# Autodesk Inventor assembly: Final Mold Assy
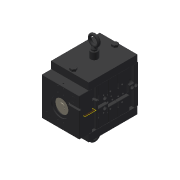
[picture p0: Inventor's stored thumbnail of the model, 180x180]
Saved by Autodesk Inventor 2022 Beta2 (Build 260130000, 130) ContinuousBuild 0
## iProperties
Shininess: 64.0
Length Units: 11269
Angle Units: 11279
Time Units: 11290
Mass Units: 11283
Length Display Precision: 3
Angle Display Precision: 2
Compacted: True
Part Number: Final Mold Assy
Document SubType Name: Assembly
Created: 2003-04-07
Designer: demo
Density: 0.0
Volumn: 0.0
Area: 0.0
PropertySet Name: Model Information
Control State: 0
Master: False
Checked Out: False
Author: demo
## Documents named in this file (9)
- C:\Autodesk Inventor 2021 Intro Practice Files\Mold Assembly\Final Mold Assy.iam
- C:\Autodesk Inventor 2021 Intro Practice Files\Mold Assembly\local.ANSI.62.230.1.ipt
- C:\Autodesk Inventor 2021 Intro Practice Files\Mold Assembly\topplate2 Assy.iam
- C:\Autodesk Inventor 2021 Intro Practice Files\Mold Assembly\Middleplate Assy.iam
- C:\Autodesk Inventor 2021 Intro Practice Files\Mold Assembly\Bottomplate2 assy1.iam
- C:\Autodesk Inventor 2021 Intro Practice Files\Mold Assembly\bottomplate.ipt
- C:\Autodesk Inventor 2021 Intro Practice Files\Mold Assembly\topplate Assy.iam
- C:\Autodesk Inventor 2021 Intro Practice Files\Mold Assembly\Sideplate.ipt
- C:\Autodesk Inventor 2021 Intro Practice Files\Mold Assembly\Grip handle.ipt
## Components (13 placed, 8 different names)
1. topplate2 Assy:1 [sub-assembly] — Mate:1, Flush:1, Mate:2, Flush:5, Flush:6, Mate:6
2. Middleplate Assy:1 [sub-assembly] — Mate:1, Flush:1, Mate:2, Flush:2, Mate:4, Mate:7, Mate:9, Flush:12
3. Bottomplate2 assy1:1 [sub-assembly] — Flush:2, Mate:4, Flush:3, Flush:4, Mate:5, Flush:12
4. topplate Assy:1 [sub-assembly] — Flush:5, Flush:6, Mate:6, Flush:7, Mate:8, Flush:9, Mate:10, Flush:10
5. Sideplate:1 — Mate:7, Flush:7, Flush:8, Mate:8, Mate:11, Insert:1, Insert:3, Insert:4
6. Grip handle:1 — Flush:8, Mate:11, Insert:1, Flush:10
7. Sideplate:2 — Mate:9, Flush:9, Mate:10, Insert:2, Flush:11, Insert:5, Insert:6
8. Grip handle:2 — Insert:2, Flush:11
9. Heavy Hex Bolt - UNC (Regular Thread - Inch) 5/8-11 UNC - 2.5:1 — Insert:3
10. Heavy Hex Bolt - UNC (Regular Thread - Inch) 5/8-11 UNC - 2.5:2 — Insert:4
11. Heavy Hex Bolt - UNC (Regular Thread - Inch) 5/8-11 UNC - 2.5:3 — Insert:5
12. Heavy Hex Bolt - UNC (Regular Thread - Inch) 5/8-11 UNC - 2.5:4 — Insert:6
13. bottomplate:1 — Flush:3, Flush:4, Mate:5
## Relationships (28: Flush 12, Mate 10, Insert 6)
- Mate:1: topplate2 Assy:1 ↔ Middleplate Assy:1
- Flush:1: topplate2 Assy:1 ↔ Middleplate Assy:1
- Mate:2: topplate2 Assy:1 ↔ Middleplate Assy:1
- Flush:2: Middleplate Assy:1 ↔ Bottomplate2 assy1:1
- Mate:4: Middleplate Assy:1 ↔ Bottomplate2 assy1:1
- Flush:3: Bottomplate2 assy1:1 ↔ bottomplate:1
- Flush:4: Bottomplate2 assy1:1 ↔ bottomplate:1
- Mate:5: Bottomplate2 assy1:1 ↔ bottomplate:1
- Flush:5: topplate2 Assy:1 ↔ topplate Assy:1
- Flush:6: topplate2 Assy:1 ↔ topplate Assy:1
- Mate:6: topplate2 Assy:1 ↔ topplate Assy:1
- Mate:7: Middleplate Assy:1 ↔ Sideplate:1
- Flush:7: topplate Assy:1 ↔ Sideplate:1
- Flush:8: Sideplate:1 ↔ Grip handle:1
- Mate:8: topplate Assy:1 ↔ Sideplate:1
- Mate:9: Middleplate Assy:1 ↔ Sideplate:2
- Flush:9: topplate Assy:1 ↔ Sideplate:2
- Mate:10: topplate Assy:1 ↔ Sideplate:2
- Mate:11: Sideplate:1 ↔ Grip handle:1
- Insert:1: Sideplate:1 ↔ Grip handle:1
- Flush:10: topplate Assy:1 ↔ Grip handle:1
- Insert:2: Sideplate:2 ↔ Grip handle:2
- Flush:11: Sideplate:2 ↔ Grip handle:2
- Insert:3: Sideplate:1 ↔ Heavy Hex Bolt - UNC (Regular Thread - Inch) 5/8-11 UNC - 2.5:1
- Insert:4: Sideplate:1 ↔ Heavy Hex Bolt - UNC (Regular Thread - Inch) 5/8-11 UNC - 2.5:2
- Insert:5: Sideplate:2 ↔ Heavy Hex Bolt - UNC (Regular Thread - Inch) 5/8-11 UNC - 2.5:3
- Insert:6: Sideplate:2 ↔ Heavy Hex Bolt - UNC (Regular Thread - Inch) 5/8-11 UNC - 2.5:4
- Flush:12: Middleplate Assy:1 ↔ Bottomplate2 assy1:1
